# Autodesk Inventor assembly: New base
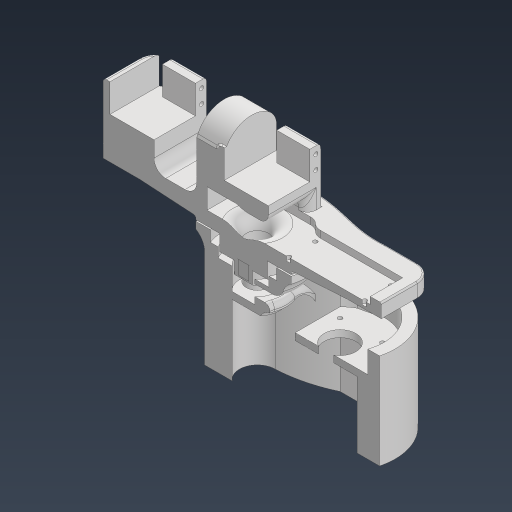
[picture p0: Inventor's stored thumbnail of the model, 512x512]
Saved by Autodesk Inventor 2024 (Build 280153000, 153)
## iProperties
Created: 2025-09-16
Part Number: New base
Document SubType Name: Assembly
Designer: Piter
Author: Piter
## Documents named in this file (4)
- C:\Users\Piter\OneDrive\Pulpit\Robots\david_Arm\Davie-Robot-Arm\3D Models\New base.iam
- C:\Users\Piter\OneDrive\Pulpit\Robots\david_Arm\Davie-Robot-Arm\3D Models\Base_v3.ipt
- C:\Users\Piter\OneDrive\Pulpit\Robots\david_Arm\Davie-Robot-Arm\3D Models\Axis1_v2.ipt
- C:\Users\Piter\OneDrive\Pulpit\Robots\david_Arm\Davie-Robot-Arm\3D Models\Gear drive.ipt
## Components (3 placed, 3 different names)
1. Base_v3:1 — Rotational:1
2. Axis1_v2:1 — Rotational:1, Rotational:2
3. Gear drive:1 — Rotational:2
## Relationships (2: RevoluteJoint 2)
- Rotational:1 [RevoluteJoint] (1 mm): Base_v3:1 ↔ Axis1_v2:1
- Rotational:2 [RevoluteJoint]: Axis1_v2:1 ↔ Gear drive:1
